# Autodesk Inventor assembly: NotchClickerAsm
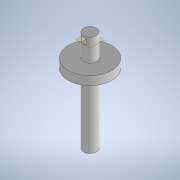
[picture p0: Inventor's stored thumbnail of the model, 180x180]
Saved by Autodesk Inventor 2021 (Build 250183000, 183)
## iProperties
Created: 2021-07-10
Part Number: NotchClickerAsm
Document SubType Name: Assembly
Designer: teh18
Author: teh18
## Documents named in this file (3)
- C:\Users\teh18\OneDrive\BVE Controller\r68-bve-mascon\NotchClickerAsm.iam
- C:\Users\teh18\OneDrive\BVE Controller\r68-bve-mascon\NotchClicker\ClickHolder.ipt
- C:\Users\teh18\OneDrive\BVE Controller\r68-bve-mascon\NotchClicker\ClickSpringBacking.ipt
## Components (2 placed, 2 different names)
1. ClickHolder:1 — Flush:1
2. ClickSpringBacking:1 — Flush:1
## Relationships (1: Flush 1)
- Flush:1: ClickHolder:1 ↔ ClickSpringBacking:1
